# Autodesk Inventor assembly: two_wheels
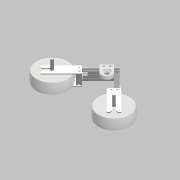
[picture p0: Inventor's stored thumbnail of the model, 180x180]
Saved by Autodesk Inventor 2021.2 (Build 252289000, 289)
## iProperties
Created: 2021-05-27
Part Number: two_wheels
Document SubType Name: Assembly
Designer: gisen
Author: gisen
## Documents named in this file (7)
- C:\Users\gisen\workspace\beetle_inventor_model\suspension\bogie.iam
- C:\Users\gisen\workspace\beetle_inventor_model\suspension\SBGSMA6904ZZ-35\SBGSMA6904ZZ-35.iam
- C:\Users\gisen\workspace\beetle_inventor_model\suspension\wheel_with_mounts.iam
- C:\Users\gisen\workspace\beetle_inventor_model\suspension\M4L.ipt
- C:\Users\gisen\workspace\beetle_inventor_model\suspension\AFS-2040-4-130.ipt
- C:\Users\gisen\workspace\beetle_inventor_model\suspension\AFS-2040-4-110.ipt
- C:\Users\gisen\workspace\beetle_inventor_model\suspension\wheel_frame_mount.ipt
## Components (8 placed, 7 different names)
1. AFS-2040-4-130:1 — メイト:1, フラッシュ:1, フラッシュ:2, 対称度:1, フラッシュ:14, フラッシュ:20, メイト:19, メイト:21
2. AFS-2040-4-110:1 — メイト:1, フラッシュ:1, フラッシュ:2, 対称度:1, メイト:22, メイト:24
3. SBGSMA6904ZZ-35:1 [sub-assembly]
4. wheel_with_mounts:1 [sub-assembly] — フラッシュ:18, 対称度:2, メイト:17, メイト:18, フラッシュ:19, メイト:23, メイト:25
5. wheel_with_mounts:2 [sub-assembly] — メイト:15, フラッシュ:18, 対称度:2, メイト:17, フラッシュ:20, メイト:20, フラッシュ:21
6. M4L:1 — メイト:19, メイト:20, メイト:21
7. wheel_frame_mount:1 — フラッシュ:21
8. bogie_mount:2 — メイト:22, メイト:23, メイト:24, メイト:25
## Relationships (30: Mate 20, Flush 7, Symmetry 2, Angle 1)
- メイト:1 [Mate]: AFS-2040-4-130:1 ↔ AFS-2040-4-110:1
- フラッシュ:1 [Flush]: AFS-2040-4-130:1 ↔ AFS-2040-4-110:1
- フラッシュ:2 [Flush]: AFS-2040-4-130:1 ↔ AFS-2040-4-110:1
- [Mate]: AFS-2040-4-130:1 ↔ SBGSMA6904ZZ-35:1
- [Angle] (0 deg): AFS-2040-4-130:1 ↔ SBGSMA6904ZZ-35:1
- [Mate]: AFS-2040-4-130:1 ↔ SBGSMA6904ZZ-35:1
- 対称度:1 [Symmetry]: AFS-2040-4-130:1 ↔ AFS-2040-4-110:1
- [Mate]: SBGSMA6904ZZ-35:1
- メイト:10 [Mate]
- メイト:11 [Mate]
- メイト:12 [Mate]
- フラッシュ:14 [Flush]: AFS-2040-4-130:1
- メイト:13 [Mate]
- メイト:14 [Mate] (200 mm)
- メイト:15 [Mate]: wheel_with_mounts:2
- フラッシュ:18 [Flush]: wheel_with_mounts:1 ↔ wheel_with_mounts:2
- 対称度:2 [Symmetry]: wheel_with_mounts:1 ↔ wheel_with_mounts:2
- メイト:16 [Mate]
- メイト:17 [Mate] (300 mm): wheel_with_mounts:1 ↔ wheel_with_mounts:2
- メイト:18 [Mate]: wheel_with_mounts:1
- フラッシュ:19 [Flush]: wheel_with_mounts:1
- フラッシュ:20 [Flush]: AFS-2040-4-130:1 ↔ wheel_with_mounts:2
- メイト:19 [Mate]: AFS-2040-4-130:1 ↔ M4L:1
- メイト:20 [Mate]: wheel_with_mounts:2 ↔ M4L:1
- メイト:21 [Mate] (-10 mm): AFS-2040-4-130:1 ↔ M4L:1
- フラッシュ:21 [Flush]: wheel_with_mounts:2 ↔ wheel_frame_mount:1
- メイト:22 [Mate]: AFS-2040-4-110:1 ↔ bogie_mount:2
- メイト:23 [Mate] (-10 mm): wheel_with_mounts:1 ↔ bogie_mount:2
- メイト:24 [Mate] (-10 mm): AFS-2040-4-110:1 ↔ bogie_mount:2
- メイト:25 [Mate] (-10 mm): wheel_with_mounts:1 ↔ bogie_mount:2
